# Autodesk Inventor assembly: A
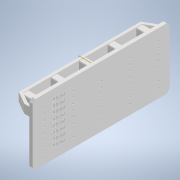
[picture p0: Inventor's stored thumbnail of the model, 180x180]
Saved by Autodesk Inventor 2022 (Build 260153000, 153)
## iProperties
Created: 2021-10-10
Part Number: A
Document SubType Name: Assembly
Designer: kfcs7
Author: kfcs7
## Documents named in this file (3)
- C:\Users\kfcs7\Desktop\Storage-Rack\A.iam
- C:\Users\kfcs7\Desktop\Storage-Rack\A-00.ipt
- C:\Users\kfcs7\Desktop\Storage-Rack\A-01.ipt
## Components (2 placed, 2 different names)
1. A-00:1 — Flush:1
2. A-01:1 — Flush:1
## Relationships (1: Flush 1)
- Flush:1: A-00:1 ↔ A-01:1
